# Autodesk Inventor assembly: potentiometer
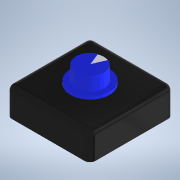
[picture p0: Inventor's stored thumbnail of the model, 180x180]
Saved by Autodesk Inventor 2020 (Build 240168000, 168)
## iProperties
Created: 2021-03-06
Part Number: potentiometer
Document SubType Name: Assembly
Designer: Harry
Author: Harry
## Documents named in this file (3)
- C:\Users\Harry\Documents\hacktheburgh\octocatch\cad\potentiometer.iam
- C:\Users\Harry\Documents\hacktheburgh\octocatch\cad\potentiometer body.ipt
- C:\Users\Harry\Documents\hacktheburgh\octocatch\cad\potentiometer knob.ipt
## Components (2 placed, 2 different names)
1. potentiometer body:1 — Insert:1
2. potentiometer knob:1 — Insert:1
## Relationships (1: Insert 1)
- Insert:1: potentiometer body:1 ↔ potentiometer knob:1
